# Autodesk Inventor assembly: Small Limit Switch
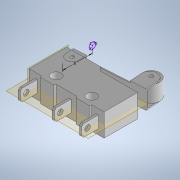
[picture p0: Inventor's stored thumbnail of the model, 180x180]
Saved by Autodesk Inventor 2020 (Build 240168000, 168)
## iProperties
Created: 2019-04-17
Part Number: Small Limit Switch
Document SubType Name: Assembly
Designer: Parker
Author: Parker
## Documents named in this file (3)
- C:\DESIGNS\MK3PRO\Extruder\Small Limit Switch\Small Limit Switch.iam
- C:\DESIGNS\MK3PRO\Extruder\Small Limit Switch\Body.ipt
- C:\DESIGNS\MK3PRO\Extruder\Small Limit Switch\Arm.ipt
## Components (2 placed, 2 different names)
1. Body:1 — Mate:1, Flush:1, Flush:2, Flush:3
2. Arm:1 — Mate:1, Flush:1, Flush:2
## Relationships (4: Flush 3, Mate 1)
- Mate:1: Body:1 ↔ Arm:1
- Flush:1: Body:1 ↔ Arm:1
- Flush:2: Body:1 ↔ Arm:1
- Flush:3 (-3.05 mm): Body:1
